# Autodesk Inventor assembly: tsop
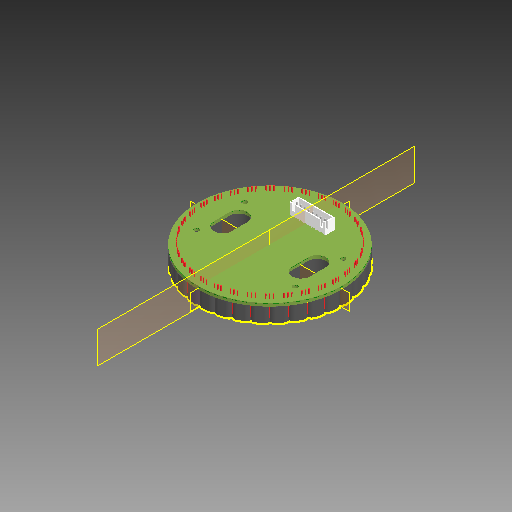
[picture p0: Inventor's stored thumbnail of the model, 512x512]
Saved by Autodesk Inventor 2020 (Build 240168000, 168)
## iProperties
Created: 2024-11-04
Part Number: tsop
Document SubType Name: Assembly
Designer: Ivan
Mass: 167.749 g
Surface Area: 509.813 cm^2
Volume: 52.0399 cm^3
Density: 3.22348 g/cm^3
Author: Ivan
## Documents named in this file (5)
- C:\!projects\DASH-\3D\Dash-V1\tsop.iam
- C:\!projects\DASH-\3D\Dash-V1\tsop_lid.ipt
- C:\!projects\DASH-\3D\Dash-V1\step\tssp58038.ipt
- C:\!projects\DASH-\3D\Dash-V1\tsop_board.ipt
- C:\!projects\DASH-\3D\Dash-V1\tssop3D\tssop3D (2).iam
## Components (35 placed, 4 different names)
1. tsop_lid:1 — Заподлицо:1, Угол:1, Угол:2, Угол:3, Совмещение:2, Совмещение:3, Совмещение:4, Совмещение:5, Вставка:1, Совмещение:7, Совмещение:8
2. tsop_board:1 — Совмещение:6, Вставка:1
3. tssop3D (2):1 [sub-assembly] — Совмещение:7, Совмещение:8
4. tssp58038:1 — Угол:1, Угол:3, Совмещение:2, Совмещение:3, Совмещение:4
5. tssp58038:2
6. tssp58038:3
7. tssp58038:4
8. tssp58038:5
9. tssp58038:6
10. tssp58038:7
11. tssp58038:8
12. tssp58038:9
13. tssp58038:10
14. tssp58038:11
15. tssp58038:12
16. tssp58038:13
17. tssp58038:14
18. tssp58038:15
19. tssp58038:16
20. tssp58038:17
21. tssp58038:18
22. tssp58038:19
23. tssp58038:20
24. tssp58038:21
25. tssp58038:22
26. tssp58038:23
27. tssp58038:24
28. tssp58038:25
29. tssp58038:26
30. tssp58038:27
31. tssp58038:28
32. tssp58038:29
33. tssp58038:30
34. tssp58038:31
35. tssp58038:32
## Component patterns: (32 elements, first: tssp58038:1)
## Relationships (12: Mate 7, Angle 3, Flush 1, Insert 1)
- Заподлицо:1 [Flush]: tsop_lid:1
- Угол:1 [Angle] (0 deg): tsop_lid:1 ↔ tssp58038:1
- Угол:2 [Angle] (0 deg): tsop_lid:1
- Угол:3 [Angle] (0 deg): tsop_lid:1 ↔ tssp58038:1
- Совмещение:2 [Mate]: tsop_lid:1 ↔ tssp58038:1
- Совмещение:3 [Mate]: tsop_lid:1 ↔ tssp58038:1
- Совмещение:4 [Mate]: tsop_lid:1 ↔ tssp58038:1
- Совмещение:5 [Mate]: tsop_lid:1
- Совмещение:6 [Mate]: tsop_board:1
- Вставка:1 [Insert]: tsop_lid:1 ↔ tsop_board:1
- Совмещение:7 [Mate]: tsop_lid:1 ↔ tssop3D (2):1
- Совмещение:8 [Mate]: tsop_lid:1 ↔ tssop3D (2):1
